# Autodesk Inventor assembly: kozepcsati2
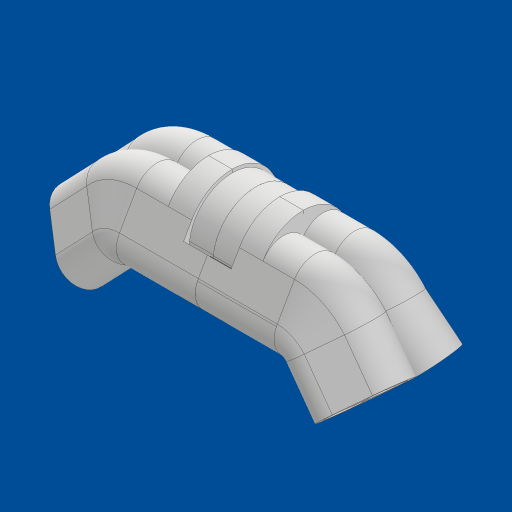
[picture p0: Inventor's stored thumbnail of the model, 512x512]
Saved by Autodesk Inventor 2023 (Build 270158000, 158)
## iProperties
Created: 2022-11-17
Part Number: kozepcsati2
Document SubType Name: Assembly
Designer: gd1
Author: gd1
## Documents named in this file (2)
- C:\Users\gd1\3D Objects\3D nagyteherbírású híd\Híd\H-d\kozepcsati2.iam
- C:\Users\gd1\3D Objects\3D nagyteherbírású híd\Híd\H-d\45 fok középcsati 2.0.ipt
## Components (2 placed, 1 different names)
1. 45 fok középcsati 2.0:1 — Insert:1
2. 45 fok középcsati 2.0:2 — Insert:1
## Relationships (1: Insert 1)
- Insert:1: 45 fok középcsati 2.0:1 ↔ 45 fok középcsati 2.0:2
